# Autodesk Inventor assembly: CIMple Box
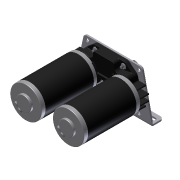
[picture p0: Inventor's stored thumbnail of the model, 180x180]
Saved by Autodesk Inventor 2011 (Build 150239000, 239)
## iProperties
Created: 2012-06-03
Part Number: CIMple Box
Document SubType Name: Assembly
Designer: Nemo
Author: Nemo
## Documents named in this file (11)
- H:\Nemo\Documents\Robotics\COTS Parts\Gearboxes\CIMple Box.iam
- H:\Nemo\Documents\Robotics\COTS Parts\Gearboxes\Housings\CIMple Box Housing.ipt
- H:\Nemo\Documents\Robotics\COTS Parts\Gearboxes\Bearings\Bearing R6zz.ipt
- H:\Nemo\Documents\Robotics\COTS Parts\Gearboxes\Shafts\CIMple Box Output Shaft.ipt
- H:\Nemo\Documents\Robotics\COTS Parts\Gearboxes\Gears\Gear 20dp 500hex 56T.ipt
- H:\Nemo\Documents\Robotics\COTS Parts\Gearboxes\Housings\CIMple Box Plate.ipt
- H:\Nemo\Documents\Robotics\COTS Parts\Gearboxes\Bearings\Bearing FR8zz.ipt
- H:\Nemo\Documents\Robotics\COTS Parts\Fasteners\10-32 SHCS x625.ipt
- H:\Nemo\Documents\Robotics\COTS Parts\Fasteners\10-32 locknut.ipt
- H:\Nemo\Documents\Robotics\COTS Parts\Motors\CIM motor 12T.iam
- H:\Nemo\Documents\Robotics\COTS Parts\Fasteners\10-32 SHCS x750.ipt
## Components (20 placed, 10 different names)
1. CIMple Box Housing:1 — Insert:1, Mate:3, Mate:4, Mate:5, Insert:8, Insert:9, Insert:10, Insert:11, Insert:12, Mate:6, Insert:13, Mate:7, Insert:14, Insert:15, Insert:16, Insert:17
2. Bearing R6zz:1 — Insert:1, Insert:2, Mate:2
3. CIMple Box Output Shaft:1 — Insert:2, Mate:1, Angle:1, Angle:2
4. Gear 56T 20dp 500hex:1 — Mate:1, Angle:1, Mate:2
5. CIMple Box Plate:1 — Insert:3, Mate:3, Mate:4, Mate:5, Insert:4, Insert:5, Insert:6, Insert:7
6. Bearing FR8zz:1 — Insert:3
7. 10-32 SHCS x625:1 — Insert:4
8. 10-32 SHCS x625:2 — Insert:5
9. 10-32 SHCS x625:3 — Insert:6
10. 10-32 SHCS x625:4 — Insert:7
11. 10-32 locknut:1 — Insert:8
12. 10-32 locknut:2 — Insert:9
13. 10-32 locknut:3 — Insert:10
14. 10-32 locknut:4 — Insert:11
15. CIM motor 12T:1 [sub-assembly] — Insert:12, Mate:6
16. CIM motor 12T:2 [sub-assembly] — Insert:13, Mate:7
17. 10-32 SHCS x750:1 — Insert:14
18. 10-32 SHCS x750:2 — Insert:15
19. 10-32 SHCS x750:3 — Insert:17
20. 10-32 SHCS x750:4 — Insert:16
## Relationships (26: Insert 17, Mate 7, Angle 2)
- Insert:1: CIMple Box Housing:1 ↔ Bearing R6zz:1
- Insert:2: Bearing R6zz:1 ↔ CIMple Box Output Shaft:1
- Mate:1: CIMple Box Output Shaft:1 ↔ Gear 56T 20dp 500hex:1
- Angle:1 (0 deg): CIMple Box Output Shaft:1 ↔ Gear 56T 20dp 500hex:1
- Mate:2: Bearing R6zz:1 ↔ Gear 56T 20dp 500hex:1
- Insert:3: CIMple Box Plate:1 ↔ Bearing FR8zz:1
- Mate:3: CIMple Box Housing:1 ↔ CIMple Box Plate:1
- Mate:4: CIMple Box Housing:1 ↔ CIMple Box Plate:1
- Mate:5: CIMple Box Housing:1 ↔ CIMple Box Plate:1
- Angle:2 (0 deg): CIMple Box Output Shaft:1
- Insert:4: CIMple Box Plate:1 ↔ 10-32 SHCS x625:1
- Insert:5: CIMple Box Plate:1 ↔ 10-32 SHCS x625:2
- Insert:6: CIMple Box Plate:1 ↔ 10-32 SHCS x625:3
- Insert:7: CIMple Box Plate:1 ↔ 10-32 SHCS x625:4
- Insert:8: CIMple Box Housing:1 ↔ 10-32 locknut:1
- Insert:9: CIMple Box Housing:1 ↔ 10-32 locknut:2
- Insert:10: CIMple Box Housing:1 ↔ 10-32 locknut:3
- Insert:11: CIMple Box Housing:1 ↔ 10-32 locknut:4
- Insert:12: CIMple Box Housing:1 ↔ CIM motor 12T:1
- Mate:6: CIMple Box Housing:1 ↔ CIM motor 12T:1
- Insert:13: CIMple Box Housing:1 ↔ CIM motor 12T:2
- Mate:7: CIMple Box Housing:1 ↔ CIM motor 12T:2
- Insert:14: CIMple Box Housing:1 ↔ 10-32 SHCS x750:1
- Insert:15: CIMple Box Housing:1 ↔ 10-32 SHCS x750:2
- Insert:16: CIMple Box Housing:1 ↔ 10-32 SHCS x750:4
- Insert:17: CIMple Box Housing:1 ↔ 10-32 SHCS x750:3
